# Autodesk Inventor assembly: Explode
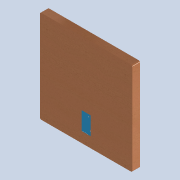
[picture p0: Inventor's stored thumbnail of the model, 180x180]
Saved by Autodesk Inventor 2021 (Build 250183000, 183)
## iProperties
Created: 2021-04-18
Part Number: Explode
Document SubType Name: Assembly
Designer: calst
Author: calst
## Documents named in this file (4)
- C:\Users\calst\OneDrive\Desktop\University Work\Year 3\Semester 2\Integrated Group Robotics Project\Group Task\AutoDesk Inventor\Explode.iam
- C:\Users\calst\OneDrive\Desktop\RFID-RC522 simple.ipt
- C:\Users\calst\OneDrive\Desktop\University Work\Year 3\Semester 2\Integrated Group Robotics Project\Group Task\AutoDesk Inventor\Board.ipt
- C:\Users\calst\OneDrive\Desktop\University Work\Year 3\Semester 2\Integrated Group Robotics Project\Group Task\AutoDesk Inventor\Playing Card RFID.ipt
## Components (3 placed, 3 different names)
1. RFID-RC522 simple:1 — Mate:1, Mate:2, Mate:3
2. Board:1 — Mate:1, Mate:2, Mate:3, Mate:4
3. Playing Card RFID:1 — Mate:4
## Relationships (4: Mate 4)
- Mate:1: RFID-RC522 simple:1 ↔ Board:1
- Mate:2: RFID-RC522 simple:1 ↔ Board:1
- Mate:3: RFID-RC522 simple:1 ↔ Board:1
- Mate:4 (0.5 mm): Board:1 ↔ Playing Card RFID:1
